# Autodesk Inventor assembly: ViaductPillar_SingleSpan-05us
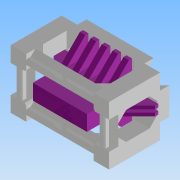
[picture p0: Inventor's stored thumbnail of the model, 180x180]
Saved by Autodesk Inventor 2021 (Build 250183000, 183)
## iProperties
Created: 2021-03-15
Part Number: ViaductPillar_SingleSpan-05us
Document SubType Name: Assembly
Designer: kumagai
Author: kumagai
## Documents named in this file (9)
- Z:\Develop\CAD\PlaRails\ViaductPillarUnit\ViaductPillar_SingleSpan.iam
- Z:\Develop\CAD\PlaRails\ViaductPillarUnit\VPU_EdgeBottom.ipt
- Z:\Develop\CAD\PlaRails\ViaductPillarUnit\VPU_EdgeTop.ipt
- Z:\Develop\CAD\PlaRails\GlobalParameter.ipt
- Z:\Develop\CAD\PlaRails\ViaductPillarUnit\VPU_SupportSingle.ipt
- ViaductPillar_SingleSpan-05u.iam
- ViaductPillar_SingleSpan-05us.iam
- ViaductPillar_SingleSpan-1u.iam
- ViaductPillar_SingleSpan-1us.iam
## Components (5 placed, 3 different names)
1. VPU_EdgeBottom:1 — メイト:1, フラッシュ:1, フラッシュ:2, フラッシュ:3, フラッシュ:4, メイト:3
2. VPU_EdgeBottom:2 — メイト:1, フラッシュ:1, フラッシュ:2
3. VPU_EdgeTop:1 — フラッシュ:3, フラッシュ:4, メイト:2, フラッシュ:5, フラッシュ:6, メイト:3
4. VPU_EdgeTop:2 — メイト:2, フラッシュ:5, フラッシュ:6
5. VPU_SupportSingle:1 — フラッシュ:7, フラッシュ:8, フラッシュ:9
## Relationships (12: Flush 9, Mate 3)
- メイト:1 [Mate]: VPU_EdgeBottom:1 ↔ VPU_EdgeBottom:2
- フラッシュ:1 [Flush]: VPU_EdgeBottom:1 ↔ VPU_EdgeBottom:2
- フラッシュ:2 [Flush]: VPU_EdgeBottom:1 ↔ VPU_EdgeBottom:2
- フラッシュ:3 [Flush]: VPU_EdgeBottom:1 ↔ VPU_EdgeTop:1
- フラッシュ:4 [Flush]: VPU_EdgeBottom:1 ↔ VPU_EdgeTop:1
- メイト:2 [Mate]: VPU_EdgeTop:1 ↔ VPU_EdgeTop:2
- フラッシュ:5 [Flush]: VPU_EdgeTop:1 ↔ VPU_EdgeTop:2
- フラッシュ:6 [Flush]: VPU_EdgeTop:1 ↔ VPU_EdgeTop:2
- メイト:3 [Mate] (-33 mm): VPU_EdgeBottom:1 ↔ VPU_EdgeTop:1
- フラッシュ:7 [Flush]: VPU_SupportSingle:1
- フラッシュ:8 [Flush]: VPU_SupportSingle:1
- フラッシュ:9 [Flush]: VPU_SupportSingle:1
## Named parameters: ViaductHeight = 66 mm, HeightRatio = 0.5, FaceShift = 0 mm
